# Autodesk Inventor assembly: OpenROV 2_2 Dev Assy
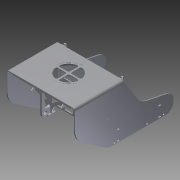
[picture p0: Inventor's stored thumbnail of the model, 180x180]
Saved by Autodesk Inventor 2011 (Build 150239000, 239)
## iProperties
Created: 2011-12-30
Part Number: OpenROV 2_2 Dev Assy
Document SubType Name: Assembly
Designer: user
Author: user
## Documents named in this file (12)
- C:\Users\user\Desktop\OpenROV\OpenROV 2.2 Dev\OpenROV 2_2 Dev Assy.iam
- C:\Users\user\Desktop\OpenROV\OpenROV 2.2 Dev\OpenROV 2_2 Dev Top.ipt
- C:\Users\user\Desktop\OpenROV\OpenROV 2.2 Dev\OpenROV 2_2 Dev Bulkhead.ipt
- C:\Users\user\Desktop\OpenROV\OpenROV 2.2 Dev\OpenROV 2_2 Dev Vertical Motor Mount.ipt
- C:\Users\user\Desktop\OpenROV\OpenROV 2.2 Dev\OpenROV 2_2 Dev Ducting Brace Mount.ipt
- C:\Users\user\Desktop\OpenROV\OpenROV 2.2 Dev\OpenROV 2_2 Dev Horizontal Motor Mount.ipt
- C:\Users\user\Desktop\OpenROV\OpenROV 2.2 Dev\OpenROV 2_2 Dev Ducting Brace.ipt
- C:\Users\user\Desktop\OpenROV\OpenROV 2.2 Dev\OpenROV 2_2 Dev Handel.ipt
- C:\Users\user\Desktop\OpenROV\OpenROV 2.2 Dev\OpenROV 2_2 Dev Ducting Separator.ipt
- C:\Users\user\Desktop\OpenROV\OpenROV 2.2 Dev\OpenROV 2_2 Dev Tube Brace.ipt
- C:\Users\user\Desktop\OpenROV\OpenROV 2.2 Dev\OpenROV 2_2 Dev Shell.ipt
- C:\Users\user\Desktop\OpenROV\OpenROV 2.2 Dev\OpenROV 2_2 Dev Prop Guard.ipt
## Components (16 placed, 11 different names)
1. OpenROV 2_2 Dev Top:1 — Mate:10, Mate:11, Flush:4, Mate:15, Mate:16, Mate:25, Mate:26, Flush:13, Flush:14, Flush:15, Mate:27, Mate:28
2. OpenROV 2_2 Dev Bulkhead:1 — Mate:7, Mate:8, Mate:9, Mate:10, Mate:11, Flush:4, Mate:23, Mate:24, Flush:16
3. OpenROV 2_2 Dev Vertical Motor Mount:1 — Mate:1, Mate:2, Mate:3, Mate:4, Flush:1, Flush:2, Flush:3
4. OpenROV 2_2 Dev Ducting Brace Mount:1 — Mate:1, Mate:4, Flush:1, Mate:5, Mate:6
5. OpenROV 2_2 Dev Ducting Brace Mount:2 — Mate:2, Mate:3, Flush:2, Mate:7, Mate:8, Mate:9, Mate:17
6. OpenROV 2_2 Dev Horizontal Motor Mount:1 — Mate:5, Mate:6, Flush:3
7. OpenROV 2_2 Dev Ducting Brace:1 — Mate:13, Flush:8, Mate:14, Mate:15, Mate:16, Mate:17, Mate:20
8. OpenROV 2_2 Dev Handel:1 — Mate:12, Flush:5, Flush:6, Flush:8, Mate:14
9. OpenROV 2_2 Dev Handel:2 — Mate:12, Flush:5, Flush:6, Mate:13, Mate:18, Mate:19
10. OpenROV 2_2 Dev Ducting Separator:1 — Mate:18, Mate:19, Mate:20
11. OpenROV 2_2 Dev Tube Brace:1 — Mate:21, Flush:9, Flush:12, Mate:23, Mate:26
12. OpenROV 2_2 Dev Tube Brace:2 — Mate:21, Flush:9, Flush:12, Flush:13
13. OpenROV 2_2 Dev Tube Brace:3 — Mate:22, Flush:10, Flush:11, Flush:14
14. OpenROV 2_2 Dev Tube Brace:4 — Mate:22, Flush:10, Flush:11, Mate:24, Mate:25
15. OpenROV 2_2 Dev Shell:1 — Flush:15, Flush:16, Mate:27, Mate:29, Mate:30
16. OpenROV 2_2 Dev Prop Guard:1 — Mate:28, Mate:29, Mate:30
## Relationships (45: Mate 30, Flush 15)
- Mate:1: OpenROV 2_2 Dev Vertical Motor Mount:1 ↔ OpenROV 2_2 Dev Ducting Brace Mount:1
- Mate:2: OpenROV 2_2 Dev Vertical Motor Mount:1 ↔ OpenROV 2_2 Dev Ducting Brace Mount:2
- Mate:3: OpenROV 2_2 Dev Vertical Motor Mount:1 ↔ OpenROV 2_2 Dev Ducting Brace Mount:2
- Mate:4: OpenROV 2_2 Dev Vertical Motor Mount:1 ↔ OpenROV 2_2 Dev Ducting Brace Mount:1
- Flush:1: OpenROV 2_2 Dev Vertical Motor Mount:1 ↔ OpenROV 2_2 Dev Ducting Brace Mount:1
- Flush:2: OpenROV 2_2 Dev Vertical Motor Mount:1 ↔ OpenROV 2_2 Dev Ducting Brace Mount:2
- Mate:5: OpenROV 2_2 Dev Ducting Brace Mount:1 ↔ OpenROV 2_2 Dev Horizontal Motor Mount:1
- Mate:6: OpenROV 2_2 Dev Ducting Brace Mount:1 ↔ OpenROV 2_2 Dev Horizontal Motor Mount:1
- Flush:3: OpenROV 2_2 Dev Vertical Motor Mount:1 ↔ OpenROV 2_2 Dev Horizontal Motor Mount:1
- Mate:7: OpenROV 2_2 Dev Bulkhead:1 ↔ OpenROV 2_2 Dev Ducting Brace Mount:2
- Mate:8: OpenROV 2_2 Dev Bulkhead:1 ↔ OpenROV 2_2 Dev Ducting Brace Mount:2
- Mate:9: OpenROV 2_2 Dev Bulkhead:1 ↔ OpenROV 2_2 Dev Ducting Brace Mount:2
- Mate:10: OpenROV 2_2 Dev Top:1 ↔ OpenROV 2_2 Dev Bulkhead:1
- Mate:11: OpenROV 2_2 Dev Top:1 ↔ OpenROV 2_2 Dev Bulkhead:1
- Flush:4: OpenROV 2_2 Dev Top:1 ↔ OpenROV 2_2 Dev Bulkhead:1
- Mate:12: OpenROV 2_2 Dev Handel:1 ↔ OpenROV 2_2 Dev Handel:2
- Flush:5: OpenROV 2_2 Dev Handel:1 ↔ OpenROV 2_2 Dev Handel:2
- Flush:6: OpenROV 2_2 Dev Handel:1 ↔ OpenROV 2_2 Dev Handel:2
- Mate:13: OpenROV 2_2 Dev Ducting Brace:1 ↔ OpenROV 2_2 Dev Handel:2
- Flush:8: OpenROV 2_2 Dev Ducting Brace:1 ↔ OpenROV 2_2 Dev Handel:1
- Mate:14: OpenROV 2_2 Dev Ducting Brace:1 ↔ OpenROV 2_2 Dev Handel:1
- Mate:15: OpenROV 2_2 Dev Top:1 ↔ OpenROV 2_2 Dev Ducting Brace:1
- Mate:16: OpenROV 2_2 Dev Top:1 ↔ OpenROV 2_2 Dev Ducting Brace:1
- Mate:17: OpenROV 2_2 Dev Ducting Brace Mount:2 ↔ OpenROV 2_2 Dev Ducting Brace:1
- Mate:18: OpenROV 2_2 Dev Handel:2 ↔ OpenROV 2_2 Dev Ducting Separator:1
- Mate:19: OpenROV 2_2 Dev Handel:2 ↔ OpenROV 2_2 Dev Ducting Separator:1
- Mate:20: OpenROV 2_2 Dev Ducting Brace:1 ↔ OpenROV 2_2 Dev Ducting Separator:1
- Mate:21: OpenROV 2_2 Dev Tube Brace:1 ↔ OpenROV 2_2 Dev Tube Brace:2
- Mate:22: OpenROV 2_2 Dev Tube Brace:3 ↔ OpenROV 2_2 Dev Tube Brace:4
- Flush:9: OpenROV 2_2 Dev Tube Brace:1 ↔ OpenROV 2_2 Dev Tube Brace:2
- Flush:10: OpenROV 2_2 Dev Tube Brace:3 ↔ OpenROV 2_2 Dev Tube Brace:4
- Flush:11: OpenROV 2_2 Dev Tube Brace:3 ↔ OpenROV 2_2 Dev Tube Brace:4
- Flush:12: OpenROV 2_2 Dev Tube Brace:1 ↔ OpenROV 2_2 Dev Tube Brace:2
- Mate:23: OpenROV 2_2 Dev Bulkhead:1 ↔ OpenROV 2_2 Dev Tube Brace:1
- Mate:24: OpenROV 2_2 Dev Bulkhead:1 ↔ OpenROV 2_2 Dev Tube Brace:4
- Mate:25: OpenROV 2_2 Dev Top:1 ↔ OpenROV 2_2 Dev Tube Brace:4
- Mate:26: OpenROV 2_2 Dev Top:1 ↔ OpenROV 2_2 Dev Tube Brace:1
- Flush:13: OpenROV 2_2 Dev Top:1 ↔ OpenROV 2_2 Dev Tube Brace:2
- Flush:14: OpenROV 2_2 Dev Top:1 ↔ OpenROV 2_2 Dev Tube Brace:3
- Flush:15: OpenROV 2_2 Dev Top:1 ↔ OpenROV 2_2 Dev Shell:1
- Flush:16: OpenROV 2_2 Dev Bulkhead:1 ↔ OpenROV 2_2 Dev Shell:1
- Mate:27: OpenROV 2_2 Dev Top:1 ↔ OpenROV 2_2 Dev Shell:1
- Mate:28: OpenROV 2_2 Dev Top:1 ↔ OpenROV 2_2 Dev Prop Guard:1
- Mate:29: OpenROV 2_2 Dev Shell:1 ↔ OpenROV 2_2 Dev Prop Guard:1
- Mate:30: OpenROV 2_2 Dev Shell:1 ↔ OpenROV 2_2 Dev Prop Guard:1
